# Autodesk Inventor assembly: robot_frame_layer1
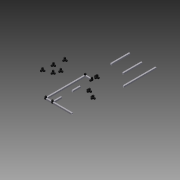
[picture p0: Inventor's stored thumbnail of the model, 180x180]
Saved by Autodesk Inventor 2011 (Build 150239000, 239)
## iProperties
Created: 2013-01-17
Part Number: robot_frame_layer1
Document SubType Name: Assembly
Designer: Christopher
Author: Christopher
## Documents named in this file (11)
- F:\Users\Christopher\Documents\GitHub\2013CAD\2013 robot\forklift\robot parts\robot_frame_layer1.iam
- F:\Users\Christopher\Documents\GitHub\2013CAD\2013 robot\forklift\robot parts\1tube_4_layer1_outside.ipt
- F:\Users\Christopher\Documents\GitHub\2013CAD\2013 robot\forklift\robot parts\1tube_6_layer1_boardsupportsupport.ipt
- F:\Users\Christopher\Documents\GitHub\2013CAD\2013 robot\forklift\robot parts\1tube_6_layer1_motorsupport.ipt
- F:\Users\Christopher\Documents\GitHub\2013CAD\2013 robot\forklift\robot parts\1tube_14_layer1_innersupport.ipt
- F:\Users\Christopher\Documents\GitHub\2013CAD\2013 robot\forklift\robot parts\1tube_14_layer1_inside.ipt
- F:\Users\Christopher\Documents\GitHub\2013CAD\2013 robot\forklift\robot parts\1tube_14_layer1_outside.ipt
- F:\Users\Christopher\Documents\GitHub\2013CAD\2013 robot\forklift\robot parts\1tube_24_layer1_outside.ipt
- F:\Users\Christopher\Documents\GitHub\2013CAD\2013 robot\forklift\robot parts\1tube_28_layer1_outside.ipt
- F:\Users\Christopher\Documents\GitHub\2013CAD\2013 robot\forklift\Misc parts\3-way corner.ipt
- F:\Users\Christopher\Documents\GitHub\2013CAD\2013 robot\forklift\Misc parts\4-way corner.ipt
## Components (21 placed, 10 different names)
1. 1tube_4_layer1_outside:1 — Mate:7, Mate:8, Mate:9, Mate:10, Mate:11, Mate:12
2. 1tube_6_layer1_boardsupportsupport:1 — Mate:22, Mate:23, Mate:24
3. 1tube_6_layer1_motorsupport:1
4. 1tube_14_layer1_innersupport:1
5. 1tube_14_layer1_inside:1
6. 1tube_14_layer1_outside:1 — Mate:19, Mate:20, Mate:21
7. 1tube_24_layer1_outside:1
8. 1tube_28_layer1_outside:1 — Mate:1, Mate:2, Mate:3, Mate:4, Mate:5, Mate:6
9. 3-way corner:1 — Mate:1, Mate:2, Mate:3, Mate:13, Mate:14, Mate:15
10. 4-way corner:1
11. 3-way corner:2 — Mate:4, Mate:5, Mate:6, Mate:7, Mate:8, Mate:9
12. 3-way corner:3
13. 3-way corner:4
14. 3-way corner:5
15. 3-way corner:6
16. 3-way corner:7 — Mate:16, Mate:17, Mate:18
17. 3-way corner:8
18. 4-way corner:2 — Mate:10, Mate:11, Mate:12, Mate:19, Mate:20, Mate:21, Mate:22, Mate:23, Mate:24
19. 1tube_4_layer1_outside:2 — Mate:13, Mate:14, Mate:15, Mate:16, Mate:17, Mate:18
20. 4-way corner:3
21. 4-way corner:4
## Relationships (24: Mate 24)
- Mate:1: 1tube_28_layer1_outside:1 ↔ 3-way corner:1
- Mate:2: 1tube_28_layer1_outside:1 ↔ 3-way corner:1
- Mate:3: 1tube_28_layer1_outside:1 ↔ 3-way corner:1
- Mate:4: 1tube_28_layer1_outside:1 ↔ 3-way corner:2
- Mate:5: 1tube_28_layer1_outside:1 ↔ 3-way corner:2
- Mate:6: 1tube_28_layer1_outside:1 ↔ 3-way corner:2
- Mate:7: 1tube_4_layer1_outside:1 ↔ 3-way corner:2
- Mate:8: 1tube_4_layer1_outside:1 ↔ 3-way corner:2
- Mate:9: 1tube_4_layer1_outside:1 ↔ 3-way corner:2
- Mate:10: 1tube_4_layer1_outside:1 ↔ 4-way corner:2
- Mate:11: 1tube_4_layer1_outside:1 ↔ 4-way corner:2
- Mate:12: 1tube_4_layer1_outside:1 ↔ 4-way corner:2
- Mate:13: 3-way corner:1 ↔ 1tube_4_layer1_outside:2
- Mate:14: 3-way corner:1 ↔ 1tube_4_layer1_outside:2
- Mate:15: 3-way corner:1 ↔ 1tube_4_layer1_outside:2
- Mate:16: 3-way corner:7 ↔ 1tube_4_layer1_outside:2
- Mate:17: 3-way corner:7 ↔ 1tube_4_layer1_outside:2
- Mate:18: 3-way corner:7 ↔ 1tube_4_layer1_outside:2
- Mate:19: 1tube_14_layer1_outside:1 ↔ 4-way corner:2
- Mate:20: 1tube_14_layer1_outside:1 ↔ 4-way corner:2
- Mate:21: 1tube_14_layer1_outside:1 ↔ 4-way corner:2
- Mate:22: 1tube_6_layer1_boardsupportsupport:1 ↔ 4-way corner:2
- Mate:23: 1tube_6_layer1_boardsupportsupport:1 ↔ 4-way corner:2
- Mate:24: 1tube_6_layer1_boardsupportsupport:1 ↔ 4-way corner:2
